# Autodesk Inventor assembly: PCB_Assembly
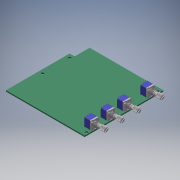
[picture p0: Inventor's stored thumbnail of the model, 180x180]
Saved by Autodesk Inventor 2017 (Build 210142000, 142)
## iProperties
Created: 2019-01-31
Part Number: PCB_Assembly
Document SubType Name: Assembly
Designer: Mitch
Author: Mitch
## Documents named in this file (3)
- E:\Youtube Channel\Pojects\Bluetooth Speaker\PCB_Assembly.iam
- E:\Youtube Channel\Pojects\Bluetooth Speaker\PCB.ipt
- E:\Youtube Channel\Pojects\Bluetooth Speaker\PTD904.ipt
## Components (5 placed, 2 different names)
1. PCB:1 — Mate:1, Mate:2, Mate:3, Mate:4, Flush:1, Flush:2, Flush:3, Flush:4, Flush:5
2. PTD904:1 — Mate:1, Flush:1, Mate:7
3. PTD904:2 — Mate:2, Flush:2, Mate:6, Mate:7
4. PTD904:3 — Mate:3, Flush:3, Mate:5, Mate:6
5. PTD904:4 — Mate:4, Flush:4, Flush:5, Mate:5
## Relationships (12: Mate 7, Flush 5)
- Mate:1: PCB:1 ↔ PTD904:1
- Mate:2: PCB:1 ↔ PTD904:2
- Mate:3: PCB:1 ↔ PTD904:3
- Mate:4: PCB:1 ↔ PTD904:4
- Flush:1: PCB:1 ↔ PTD904:1
- Flush:2: PCB:1 ↔ PTD904:2
- Flush:3: PCB:1 ↔ PTD904:3
- Flush:4: PCB:1 ↔ PTD904:4
- Flush:5 (10.414 mm): PCB:1 ↔ PTD904:4
- Mate:5 (21.3614 mm): PTD904:3 ↔ PTD904:4
- Mate:6 (12.065 mm): PTD904:2 ↔ PTD904:3
- Mate:7 (12.065 mm): PTD904:1 ↔ PTD904:2
